# Autodesk Inventor assembly: coupler extention arm collector middle + pulleys
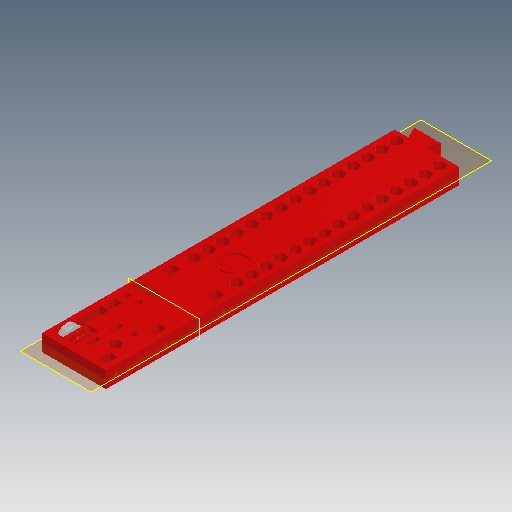
[picture p0: Inventor's stored thumbnail of the model, 512x512]
Saved by Autodesk Inventor 2020 (Build 240168000, 168)
## iProperties
Created: 2020-01-01
Part Number: coupler extention arm collector middle + pulleys
Document SubType Name: Assembly
Designer: ball
Author: ball
## Documents named in this file (4)
- C:\FTC\FTC8863CAD\2019 Robot\Delivery\extension arm\coupler extention arm collector middle + pulleys.iam
- C:\FTC\FTC8863CAD\2019 Robot\Delivery\extension arm\Coupler extension arm short.ipt
- C:\FTC\FTC8863CAD\RevRobotics\REV-41-1368 pulley.ipt
- C:\FTC\FTC8863CAD\2019 Robot\Delivery\plastic pulley deep u.ipt
## Components (3 placed, 3 different names)
1. Coupler extension arm short:1 — Mate:1, Mate:2, Mate:5, Mate:6
2. REV-41-1368 pulley:1 — Mate:1, Mate:2
3. plastic pulley deep u:1 — Mate:5, Mate:6
## Relationships (4: Mate 4)
- Mate:1: Coupler extension arm short:1 ↔ REV-41-1368 pulley:1
- Mate:2: Coupler extension arm short:1 ↔ REV-41-1368 pulley:1
- Mate:5: Coupler extension arm short:1 ↔ plastic pulley deep u:1
- Mate:6: Coupler extension arm short:1 ↔ plastic pulley deep u:1
